# Autodesk Inventor assembly: Ensamblaje2
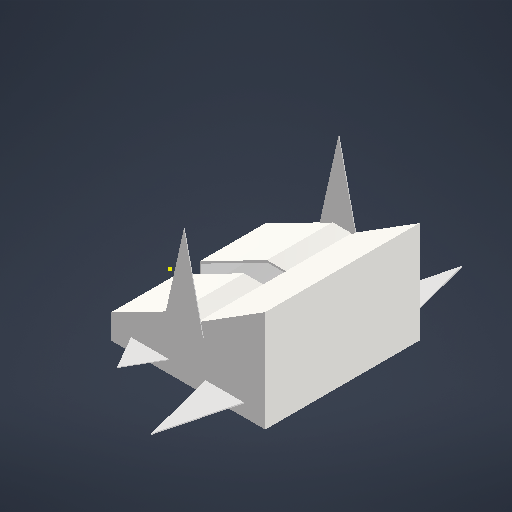
[picture p0: Inventor's stored thumbnail of the model, 512x512]
Saved by Autodesk Inventor 2027 (Build 310192060, 192F)
## iProperties
Created: 2026-08-23
Part Number: Ensamblaje2
Document SubType Name: Assembly
Designer: Leandro
Finish3_Appearance: Aluminum - Polished
Finish3_Area: 373937.644 mm^2
Author: Leandro
## Documents named in this file (5)
- C:\Users\Leandro\Desktop\Ensamblaje2.iam
- C:\Users\Leandro\Desktop\lateral triangular .ipt
- C:\Users\Leandro\Desktop\Pieza2.ipt
- C:\Users\Leandro\Desktop\Pieza3.ipt
- C:\Users\Leandro\Desktop\Pieza4.ipt
## Components (7 placed, 4 different names)
1. lateral triangular :1 — Coincidencia:1, Coincidencia:2, Coincidencia:3, Coincidencia:4, Coincidencia:5, Coincidencia:6
2. Pieza2:1 — Coincidencia:1
3. Pieza2:2 — Coincidencia:2
4. Pieza3:1 — Coincidencia:3
5. Pieza3:2 — Coincidencia:4
6. Pieza4:1 — Coincidencia:5
7. Pieza4:2 — Coincidencia:6
## Relationships (6: Mate 6)
- Coincidencia:1 [Mate]: lateral triangular :1 ↔ Pieza2:1
- Coincidencia:2 [Mate]: lateral triangular :1 ↔ Pieza2:2
- Coincidencia:3 [Mate]: lateral triangular :1 ↔ Pieza3:1
- Coincidencia:4 [Mate]: lateral triangular :1 ↔ Pieza3:2
- Coincidencia:5 [Mate]: lateral triangular :1 ↔ Pieza4:1
- Coincidencia:6 [Mate]: lateral triangular :1 ↔ Pieza4:2
## Named parameters: Finish1_Area = 4150.59, Finish2_Area = 7087.1, Finish3_Area = 3739.38
note: some values were not read from the file. Shown as the stored number, unit unknown: "Finish1_Area", "Finish2_Area", "Finish3_Area".
